# Autodesk Inventor assembly: Luftverteiler
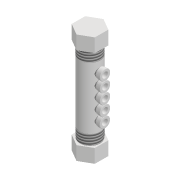
[picture p0: Inventor's stored thumbnail of the model, 180x180]
Saved by Autodesk Inventor 2021 (Build 250183000, 183)
## iProperties
Created: 2022-02-28
Part Number: Luftverteiler
Document SubType Name: Assembly
Designer: lukas
Author: lukas
## Documents named in this file (4)
- C:\Users\lukas\OneDrive - HTBLA Kaindorf\Diplomarbeit\Mechanik\InventorKonstruktion\Luftverteiler.iam
- C:\Users\lukas\OneDrive - HTBLA Kaindorf\Diplomarbeit\Mechanik\InventorKonstruktion\VerteilerLuft1.ipt
- C:\Users\lukas\OneDrive - HTBLA Kaindorf\Diplomarbeit\Mechanik\InventorKonstruktion\VerteilerLuft2.ipt
- C:\Users\lukas\OneDrive - HTBLA Kaindorf\Diplomarbeit\Mechanik\InventorKonstruktion\Schlauchsteckverbindung.ipt
## Components (8 placed, 3 different names)
1. VerteilerLuft1:1 — Zylindrisch:1, Passend:1, Zylindrisch:2, Passend:2, Starr:1, Starr:2, Starr:3, Starr:4, Starr:5
2. VerteilerLuft2:1 — Zylindrisch:1, Passend:1
3. VerteilerLuft2:2 — Zylindrisch:2, Passend:2
4. Schlauchsteckverbindung:1 — Starr:2
5. Schlauchsteckverbindung:2 — Starr:3
6. Schlauchsteckverbindung:3 — Starr:4
7. Schlauchsteckverbindung:4 — Starr:1
8. Schlauchsteckverbindung:5 — Starr:5
## Relationships (9: WeldJoint 5, CylindricalJoint 2, Mate 2)
- Zylindrisch:1 [CylindricalJoint]: VerteilerLuft1:1 ↔ VerteilerLuft2:1
- Passend:1 [Mate] (-10 mm): VerteilerLuft1:1 ↔ VerteilerLuft2:1
- Zylindrisch:2 [CylindricalJoint]: VerteilerLuft1:1 ↔ VerteilerLuft2:2
- Passend:2 [Mate] (-10 mm): VerteilerLuft1:1 ↔ VerteilerLuft2:2
- Starr:1 [WeldJoint] (5 mm): VerteilerLuft1:1 ↔ Schlauchsteckverbindung:4
- Starr:2 [WeldJoint] (-7 mm): VerteilerLuft1:1 ↔ Schlauchsteckverbindung:1
- Starr:3 [WeldJoint] (-7 mm): VerteilerLuft1:1 ↔ Schlauchsteckverbindung:2
- Starr:4 [WeldJoint] (-7 mm): VerteilerLuft1:1 ↔ Schlauchsteckverbindung:3
- Starr:5 [WeldJoint] (-7 mm): VerteilerLuft1:1 ↔ Schlauchsteckverbindung:5
